# Autodesk Inventor assembly: x_passive
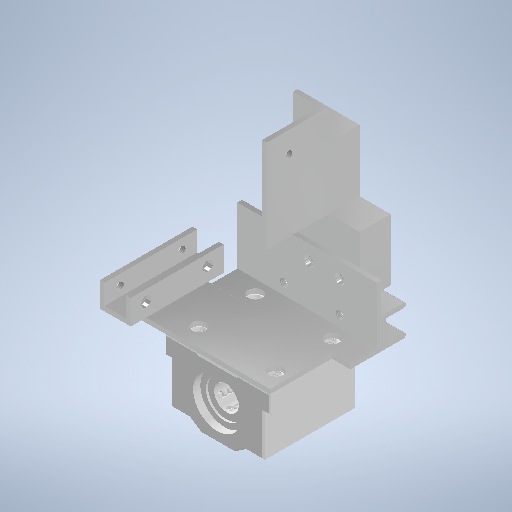
[picture p0: Inventor's stored thumbnail of the model, 512x512]
Saved by Autodesk Inventor 2025 (Build 290162000, 162)
## iProperties
Created: 2024-04-25
Part Number: x_passive
Document SubType Name: Assembly
Designer: rader
Author: rader
## Documents named in this file (7)
- C:\Users\rader\Documents\rp\x_passive.iam
- C:\Users\rader\Documents\rp\y_bearing.ipt
- C:\Users\rader\Documents\rp\x_bracket.ipt
- C:\Users\rader\Documents\rp\x_holder.ipt
- C:\Users\rader\Documents\rp\x_bearing_tab.ipt
- C:\Users\rader\Documents\rp\y_anchor_holder.ipt
- C:\Users\rader\Documents\rp\y_belt_anchor.ipt
## Components (6 placed, 6 different names)
1. y_bearing:1 — Proti sobě:1, Stejný směr:1, Stejný směr:2, Proti sobě:2, Stejný směr:3, Stejný směr:4, Proti sobě:4, Stejný směr:5
2. x_bracket:1 — Proti sobě:2, Stejný směr:3, Stejný směr:4, Vložit:1, Vložit:2, Vložit:3, Vložit:4, Proti sobě:3
3. x_holder:1 — Vložit:1, Vložit:2
4. x_bearing_tab:1 — Vložit:3, Vložit:4
5. y_anchor_holder:1 — Proti sobě:3, Proti sobě:4, Stejný směr:5, Vložit:5, Stejný směr:6
6. y_belt_anchor:1 — Vložit:5, Stejný směr:6
## Relationships (15: Flush 6, Insert 5, Mate 4)
- Proti sobě:1 [Mate]: y_bearing:1
- Stejný směr:1 [Flush]: y_bearing:1
- Stejný směr:2 [Flush]: y_bearing:1
- Proti sobě:2 [Mate]: y_bearing:1 ↔ x_bracket:1
- Stejný směr:3 [Flush]: y_bearing:1 ↔ x_bracket:1
- Stejný směr:4 [Flush] (-6 mm): y_bearing:1 ↔ x_bracket:1
- Vložit:1 [Insert]: x_bracket:1 ↔ x_holder:1
- Vložit:2 [Insert]: x_bracket:1 ↔ x_holder:1
- Vložit:3 [Insert]: x_bracket:1 ↔ x_bearing_tab:1
- Vložit:4 [Insert]: x_bracket:1 ↔ x_bearing_tab:1
- Proti sobě:3 [Mate]: x_bracket:1 ↔ y_anchor_holder:1
- Proti sobě:4 [Mate]: y_bearing:1 ↔ y_anchor_holder:1
- Stejný směr:5 [Flush]: y_bearing:1 ↔ y_anchor_holder:1
- Vložit:5 [Insert]: y_anchor_holder:1 ↔ y_belt_anchor:1
- Stejný směr:6 [Flush]: y_anchor_holder:1 ↔ y_belt_anchor:1
